# Autodesk Inventor assembly: HbHand
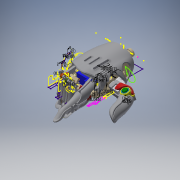
[picture p0: Inventor's stored thumbnail of the model, 180x180]
Saved by Autodesk Inventor 2017 (Build 210142000, 142)
## iProperties
Part Number: HbHand
Material: 一般
Document SubType Name: Assembly
Designer: sktom
Author: sktom
## Documents named in this file (20)
- D:\OneDrive\CAD\MAJ\hackberry\HACKberry-hardware\3D_69%inlength\Inventor\HbHandForChild\HbHand.iam
- D:\OneDrive\CAD\MAJ\hackberry\HACKberry-hardware\3D_69%inlength\Inventor\HbHandForChild\HbPalmBase03ForChild.ipt
- D:\OneDrive\CAD\MAJ\hackberry\HACKberry-hardware\3D_69%inlength\Inventor\HbHandForChild\bearing_683.ipt
- D:\OneDrive\CAD\MAJ\hackberry\HACKberry-hardware\3D_69%inlength\Inventor\HbHandForChild\HbthumbU02ForChild\HbthumbU02ForChild.iam
- D:\OneDrive\CAD\MAJ\hackberry\HACKberry-hardware\3D_69%inlength\Inventor\HbHandForChild\HbServoHK282A\Servo_HK282A_Hone.ipt
- D:\OneDrive\CAD\MAJ\hackberry\HACKberry-hardware\3D_69%inlength\Inventor\HbHandForChild\HbIndexFinger01ForChild\HbIndexFinger01ForChild.iam
- D:\OneDrive\CAD\MAJ\hackberry\HACKberry-hardware\3D_69%inlength\Inventor\HbHandForChild\HbFinger01ForChild\HbFinger01ForChild.iam
- D:\OneDrive\CAD\MAJ\hackberry\HACKberry-hardware\3D_69%inlength\Inventor\HbHandForChild\HbRing-LittleCouplerLink01ForChild.ipt
- D:\OneDrive\CAD\MAJ\hackberry\HACKberry-hardware\3D_69%inlength\Inventor\HbHandForChild\HbMiddle-RingCouplerLink01ForChild.ipt
- D:\OneDrive\CAD\MAJ\hackberry\HACKberry-hardware\3D_69%inlength\Inventor\HbHandForChild\servo\Tower Pro 9g Micro Servo SG90.iam
- D:\OneDrive\CAD\MAJ\hackberry\HACKberry-hardware\3D_69%inlength\Inventor\HbHandForChild\DummyASV-15MG.ipt
- D:\OneDrive\CAD\MAJ\hackberry\HACKberry-hardware\3D_69%inlength\Inventor\HbHandForChild\HbFingerMainCouplerLink01ForChild.ipt
- D:\OneDrive\CAD\MAJ\hackberry\HACKberry-hardware\3D_69%inlength\Inventor\HbHandForChild\DummyASV-15MGSingleHorn01.ipt
- D:\OneDrive\CAD\MAJ\hackberry\HACKberry-hardware\3D_69%inlength\Inventor\HbHandForChild\HbBackCover02ForChild.ipt
- D:\OneDrive\CAD\MAJ\hackberry\HACKberry-hardware\3D_69%inlength\Inventor\HbHandForChild\Spur Gear (16 teeth).ipt
- D:\OneDrive\CAD\MAJ\hackberry\HACKberry-hardware\3D_69%inlength\Inventor\HbHandForChild\spacer_2_3_l3.5.ipt
- D:\OneDrive\CAD\MAJ\hackberry\HACKberry-hardware\3D_69%inlength\Inventor\HbHandForChild\HbServoCover.ipt
- D:\OneDrive\CAD\MAJ\hackberry\HACKberry-hardware\3D_69%inlength\Inventor\HbHandForChild\HbShaftStopperB04ForChild.ipt
- D:\OneDrive\CAD\MAJ\hackberry\HACKberry-hardware\3D_69%inlength\Inventor\HbHandForChild\HbShaftStopperA04ForChild.ipt
- D:\OneDrive\CAD\MAJ\hackberry\HACKberry-hardware\3D_69%inlength\Inventor\HbHandForChild\shaft_phi1.5_l10.ipt
## Components (32 placed, 19 different names)
1. HbPalmBase03ForChild:1 — 挿入:1, 挿入:4, 挿入:5, 挿入:6, 挿入:7, 挿入:8, 挿入:9, 挿入:10, 挿入:11, 挿入:12, 挿入:15, 挿入:16, メイト:2, メイト:3, 挿入:22, 挿入:23, 挿入:31, 挿入:32, 挿入:33, 挿入:34, 挿入:35, 挿入:36, 挿入:37, 挿入:38, 挿入:39, 挿入:40, 挿入:41
2. bearing_683:1 — 挿入:1, 挿入:2
3. HbthumbU02ForChild:1 [sub-assembly] — 挿入:2, 挿入:3
4. Servo_HK282A_Hone:1 — 挿入:3, 挿入:4, 挿入:5
5. HbIndexFinger01ForChild:1 [sub-assembly] — 挿入:6
6. HbFinger01ForChild:1 [sub-assembly] — 挿入:7, 挿入:8, 挿入:13, 挿入:30
7. HbFinger01ForChild:2 [sub-assembly] — 挿入:9, 挿入:10, 円柱状:1, 挿入:14, 挿入:28, 挿入:29
8. HbFinger01ForChild:3 [sub-assembly] — 挿入:11, 挿入:12, 円柱状:2, 挿入:19, 挿入:26, 挿入:27
9. HbRing-LittleCouplerLink01ForChild:1 — 挿入:14, 円柱状:2
10. HbMiddle-RingCouplerLink01ForChild:1 — 挿入:13, 円柱状:1
11. Tower Pro 9g Micro Servo SG90:1 [sub-assembly] — 挿入:15, 挿入:16, 挿入:24
12. DummyASV-15MG:1 — 挿入:20, メイト:2, メイト:3
13. HbFingerMainCouplerLink01ForChild:1 — 挿入:19, 挿入:42, 挿入:43
14. DummyASV-15MGSingleHorn01:1 — 挿入:20, 挿入:42
15. HbBackCover02ForChild:1 — 挿入:22, 挿入:23
16. Spur Gear (16 teeth):1 — 挿入:24
17. spacer_2_3_l3.5:1 — 挿入:26
18. spacer_2_3_l3.5:2 — 挿入:43
19. spacer_2_3_l3.5:3 — 挿入:27
20. spacer_2_3_l3.5:4 — 挿入:28
21. spacer_2_3_l3.5:5 — 挿入:29
22. spacer_2_3_l3.5:6 — 挿入:30
23. HbServoCover:1 — 挿入:31, 挿入:32
24. HbShaftStopperB04ForChild:1 — 挿入:34
25. HbShaftStopperA04ForChild:1 — 挿入:33
26. shaft_phi1.5_l10:1 — 挿入:35
27. shaft_phi1.5_l10:2 — 挿入:36
28. shaft_phi1.5_l10:3 — 挿入:37
29. shaft_phi1.5_l10:4 — 挿入:38
30. shaft_phi1.5_l10:5 — 挿入:39
31. shaft_phi1.5_l10:6 — 挿入:41
32. shaft_phi1.5_l10:7 — 挿入:40
## Relationships (43: Insert 39, CylindricalJoint 2, Mate 2)
- 挿入:1 [Insert]: HbPalmBase03ForChild:1 ↔ bearing_683:1
- 挿入:2 [Insert]: bearing_683:1 ↔ HbthumbU02ForChild:1
- 挿入:3 [Insert]: HbthumbU02ForChild:1 ↔ Servo_HK282A_Hone:1
- 挿入:4 [Insert]: HbPalmBase03ForChild:1 ↔ Servo_HK282A_Hone:1
- 挿入:5 [Insert]: HbPalmBase03ForChild:1 ↔ Servo_HK282A_Hone:1
- 挿入:6 [Insert]: HbPalmBase03ForChild:1 ↔ HbIndexFinger01ForChild:1
- 挿入:7 [Insert]: HbPalmBase03ForChild:1 ↔ HbFinger01ForChild:1
- 挿入:8 [Insert]: HbPalmBase03ForChild:1 ↔ HbFinger01ForChild:1
- 挿入:9 [Insert]: HbPalmBase03ForChild:1 ↔ HbFinger01ForChild:2
- 挿入:10 [Insert]: HbPalmBase03ForChild:1 ↔ HbFinger01ForChild:2
- 挿入:11 [Insert]: HbPalmBase03ForChild:1 ↔ HbFinger01ForChild:3
- 挿入:12 [Insert]: HbPalmBase03ForChild:1 ↔ HbFinger01ForChild:3
- 挿入:13 [Insert]: HbFinger01ForChild:1 ↔ HbMiddle-RingCouplerLink01ForChild:1
- 円柱状:1 [CylindricalJoint]: HbFinger01ForChild:2 ↔ HbMiddle-RingCouplerLink01ForChild:1
- 挿入:14 [Insert]: HbFinger01ForChild:2 ↔ HbRing-LittleCouplerLink01ForChild:1
- 円柱状:2 [CylindricalJoint]: HbFinger01ForChild:3 ↔ HbRing-LittleCouplerLink01ForChild:1
- 挿入:15 [Insert]: HbPalmBase03ForChild:1 ↔ Tower Pro 9g Micro Servo SG90:1
- 挿入:16 [Insert]: HbPalmBase03ForChild:1 ↔ Tower Pro 9g Micro Servo SG90:1
- 挿入:19 [Insert] (0.1 mm): HbFinger01ForChild:3 ↔ HbFingerMainCouplerLink01ForChild:1
- 挿入:20 [Insert]: DummyASV-15MG:1 ↔ DummyASV-15MGSingleHorn01:1
- メイト:2 [Mate]: HbPalmBase03ForChild:1 ↔ DummyASV-15MG:1
- メイト:3 [Mate]: HbPalmBase03ForChild:1 ↔ DummyASV-15MG:1
- 挿入:22 [Insert]: HbPalmBase03ForChild:1 ↔ HbBackCover02ForChild:1
- 挿入:23 [Insert]: HbPalmBase03ForChild:1 ↔ HbBackCover02ForChild:1
- 挿入:24 [Insert] (0.8 mm): Tower Pro 9g Micro Servo SG90:1 ↔ Spur Gear (16 teeth):1
- 挿入:26 [Insert]: HbFinger01ForChild:3 ↔ spacer_2_3_l3.5:1
- 挿入:27 [Insert]: HbFinger01ForChild:3 ↔ spacer_2_3_l3.5:3
- 挿入:28 [Insert]: HbFinger01ForChild:2 ↔ spacer_2_3_l3.5:4
- 挿入:29 [Insert]: HbFinger01ForChild:2 ↔ spacer_2_3_l3.5:5
- 挿入:30 [Insert]: HbFinger01ForChild:1 ↔ spacer_2_3_l3.5:6
- 挿入:31 [Insert]: HbPalmBase03ForChild:1 ↔ HbServoCover:1
- 挿入:32 [Insert]: HbPalmBase03ForChild:1 ↔ HbServoCover:1
- 挿入:33 [Insert]: HbPalmBase03ForChild:1 ↔ HbShaftStopperA04ForChild:1
- 挿入:34 [Insert]: HbPalmBase03ForChild:1 ↔ HbShaftStopperB04ForChild:1
- 挿入:35 [Insert]: HbPalmBase03ForChild:1 ↔ shaft_phi1.5_l10:1
- 挿入:36 [Insert] (0.5 mm): HbPalmBase03ForChild:1 ↔ shaft_phi1.5_l10:2
- 挿入:37 [Insert] (0.3 mm): HbPalmBase03ForChild:1 ↔ shaft_phi1.5_l10:3
- 挿入:38 [Insert] (0.3 mm): HbPalmBase03ForChild:1 ↔ shaft_phi1.5_l10:4
- 挿入:39 [Insert] (0.5 mm): HbPalmBase03ForChild:1 ↔ shaft_phi1.5_l10:5
- 挿入:40 [Insert] (0.5 mm): HbPalmBase03ForChild:1 ↔ shaft_phi1.5_l10:7
- 挿入:41 [Insert] (0.5 mm): HbPalmBase03ForChild:1 ↔ shaft_phi1.5_l10:6
- 挿入:42 [Insert]: HbFingerMainCouplerLink01ForChild:1 ↔ DummyASV-15MGSingleHorn01:1
- 挿入:43 [Insert]: HbFingerMainCouplerLink01ForChild:1 ↔ spacer_2_3_l3.5:2
